# Autodesk Inventor assembly: Assembly_smooth
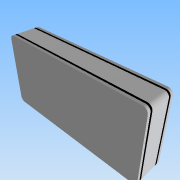
[picture p0: Inventor's stored thumbnail of the model, 180x180]
Saved by Autodesk Inventor 2016 (Build 200138000, 138)
## iProperties
Created: 2015-09-13
Part Number: Assembly_smooth
Document SubType Name: Assembly
Designer: Openlab
Author: Openlab
## Documents named in this file (11)
- D:\Alexey\HS-Spectrophotometer\parts\Paris\Assembly_smooth.iam
- D:\Alexey\HS-Spectrophotometer\parts\Paris\Box2_walls.ipt
- D:\Alexey\HS-Spectrophotometer\parts\Paris\Box2_top.ipt
- D:\Alexey\HS-Spectrophotometer\parts\Paris\Box2_spacer.ipt
- D:\Alexey\HS-Spectrophotometer\parts\Paris\Core_bottom-im.ipt
- D:\Alexey\HS-Spectrophotometer\parts\Paris\Core_top-im.ipt
- D:\Alexey\HS-Spectrophotometer\parts\Common\LCD5110.ipt
- D:\Alexey\HS-Spectrophotometer\parts\Paris\Box2_bottom.ipt
- D:\Alexey\HS-Spectrophotometer\parts\Common\LCD12864-large.ipt
- D:\Alexey\HS-Spectrophotometer\parts\Common\LCD12864-large-film.ipt
- D:\Alexey\HS-Spectrophotometer\parts\Common\Cuvette.ipt
## Components (11 placed, 10 different names)
1. Box2_walls:1 — Mate:2, Mate:3, Mate:6, Mate:19, Flush:21, Flush:22, Mate:20, Mate:21, Mate:22
2. Box2_top:1 — Mate:2, Mate:3, Mate:4, Mate:5, Mate:14, Mate:15, Mate:16, Mate:17, Mate:23, Mate:28, Mate:29, Flush:29, Mate:30
3. Box2_spacer:1 — Mate:4, Mate:5, Mate:6, Mate:30
4. Core_bottom-im:1 — Mate:7, Mate:8, Mate:9, Mate:34, Mate:35, Mate:36
5. Core_top-im:1 — Mate:7, Mate:8, Mate:9, Mate:14, Mate:15, Flush:29
6. LCD5110:1 — Mate:16, Mate:17
7. Box2_spacer:2 — Mate:19, Flush:21, Flush:22
8. Box2_bottom:1 — Mate:20, Mate:21, Mate:22
9. LCD12864-large:2 — Mate:23, Mate:27, Flush:28, Mate:28, Mate:29, Flush:30
10. LCD12864-large-film:1 — Mate:27, Flush:28, Flush:30
11. Cuvette:1 — Mate:34, Mate:35, Mate:36
## Relationships (29: Mate 24, Flush 5)
- Mate:2: Box2_walls:1 ↔ Box2_top:1
- Mate:3: Box2_walls:1 ↔ Box2_top:1
- Mate:4: Box2_top:1 ↔ Box2_spacer:1
- Mate:5: Box2_top:1 ↔ Box2_spacer:1
- Mate:6: Box2_walls:1 ↔ Box2_spacer:1
- Mate:7: Core_bottom-im:1 ↔ Core_top-im:1
- Mate:8: Core_bottom-im:1 ↔ Core_top-im:1
- Mate:9: Core_bottom-im:1 ↔ Core_top-im:1
- Mate:14: Box2_top:1 ↔ Core_top-im:1
- Mate:15: Box2_top:1 ↔ Core_top-im:1
- Mate:16: Box2_top:1 ↔ LCD5110:1
- Mate:17: Box2_top:1 ↔ LCD5110:1
- Mate:19: Box2_walls:1 ↔ Box2_spacer:2
- Flush:21: Box2_walls:1 ↔ Box2_spacer:2
- Flush:22: Box2_walls:1 ↔ Box2_spacer:2
- Mate:20: Box2_walls:1 ↔ Box2_bottom:1
- Mate:21: Box2_walls:1 ↔ Box2_bottom:1
- Mate:22: Box2_walls:1 ↔ Box2_bottom:1
- Mate:23: Box2_top:1 ↔ LCD12864-large:2
- Mate:27: LCD12864-large:2 ↔ LCD12864-large-film:1
- Flush:28: LCD12864-large:2 ↔ LCD12864-large-film:1
- Mate:28: Box2_top:1 ↔ LCD12864-large:2
- Mate:29: Box2_top:1 ↔ LCD12864-large:2
- Flush:29: Box2_top:1 ↔ Core_top-im:1
- Mate:30: Box2_top:1 ↔ Box2_spacer:1
- Flush:30: LCD12864-large:2 ↔ LCD12864-large-film:1
- Mate:34: Core_bottom-im:1 ↔ Cuvette:1
- Mate:35: Core_bottom-im:1 ↔ Cuvette:1
- Mate:36: Core_bottom-im:1 ↔ Cuvette:1
